# Autodesk Inventor assembly: mainAsm-mainAsm
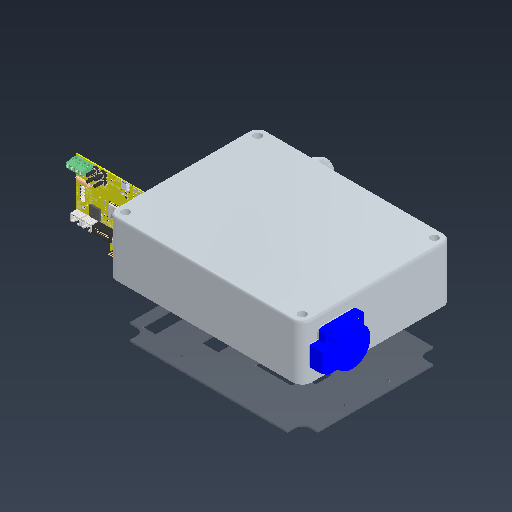
[picture p0: Inventor's stored thumbnail of the model, 512x512]
Saved by Autodesk Inventor 2026.2 (Build 302298000, 298)
## iProperties
Created: 2026-03-04
Part Number: mainAsm-mainAsm
Description: FreeCAD Model
Document SubType Name: Assembly
Designer: MenMe
Authority: Unknown
Title: Open CASCADE Shape Model
Sending System: FreeCAD
Preprocessor: Open CASCADE STEP processor 7.8
## Documents named in this file (18)
- C:\Users\MenMe\Downloads\mainAsm-mainAsm\mainAsm-mainAsm\mainAsm-mainAsm.iam
- C:\Users\MenMe\Downloads\mainAsm-mainAsm\mainAsm-mainAsm\Main box.iam
- C:\Users\MenMe\Downloads\mainAsm-mainAsm\mainAsm-mainAsm\DIN rail.iam
- C:\Users\MenMe\Downloads\mainAsm-mainAsm\mainAsm-mainAsm\DIN rail_1.iam
- C:\Users\MenMe\Downloads\mainAsm-mainAsm\mainAsm-mainAsm\Breaker.iam
- C:\Users\MenMe\Downloads\mainAsm-mainAsm\mainAsm-mainAsm\source24V.ipt
- C:\Users\MenMe\Downloads\mainAsm-mainAsm\mainAsm-mainAsm\source5V.ipt
- C:\Users\MenMe\Downloads\mainAsm-mainAsm\mainAsm-mainAsm\Relay.ipt
- C:\Users\MenMe\Downloads\mainAsm-mainAsm\mainAsm-mainAsm\Measuring Asm.iam
- C:\Users\MenMe\Downloads\mainAsm-mainAsm\mainAsm-mainAsm\Passthrough.ipt
- C:\Users\MenMe\Downloads\mainAsm-mainAsm\mainAsm-mainAsm\Gasket.ipt
- C:\Users\MenMe\Downloads\mainAsm-mainAsm\mainAsm-mainAsm\Ring Nut.ipt
- C:\Users\MenMe\Downloads\mainAsm-mainAsm\mainAsm-mainAsm\Socket.ipt
- C:\Users\MenMe\Downloads\mainAsm-mainAsm\mainAsm-mainAsm\Gasket_1.ipt
- C:\Users\MenMe\Downloads\mainAsm-mainAsm\mainAsm-mainAsm\fuseHolder.iam
- C:\Users\MenMe\Downloads\mainAsm-mainAsm\mainAsm-mainAsm\pcbAsm2.iam
- C:\Users\MenMe\Downloads\mainAsm-mainAsm\mainAsm-mainAsm\Body_2.ipt
- C:\Users\MenMe\Documents\GitHub\SchoolStuff\rose\rose_pcb\rose_pcb\rose_pcb.iam
## Components (18 placed, 18 different names)
1. 2 [sub-assembly] — Mate:1, Mate:2
2. 4 [sub-assembly]
3. 5 [sub-assembly]
4. 7 [sub-assembly]
5. 9 [sub-assembly]
6. 10
7. 11
8. 12
9. 24 [sub-assembly]
10. 25
11. 26
12. 27
13. 28
14. 29
15. 32 [sub-assembly]
16. 45 [sub-assembly]
17. 46 — Mate:1, Mate:2
18. rose_pcb:1 [sub-assembly]
## Relationships (2: Mate 2)
- Mate:1: 2 ↔ 46
- Mate:2: 2 ↔ 46
